# Autodesk Inventor assembly: BP-100
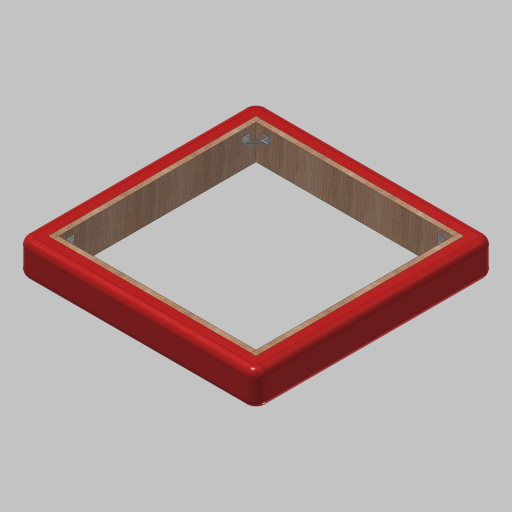
[picture p0: Inventor's stored thumbnail of the model, 512x512]
Saved by Autodesk Inventor 2023.5 (Build 275446000, 446)
## iProperties
Created: 2025-01-26
Part Number: BP-100
Document SubType Name: Assembly
Designer: slick
Author: slick
## Documents named in this file (5)
- C:\Users\slick\OneDrive\Desktop\2025-ReefScape---CAD\Bumpers\BP-100.iam
- C:\Users\slick\OneDrive\Desktop\2025-ReefScape---CAD\Bumpers\BP-001.ipt
- C:\Users\slick\OneDrive\Desktop\2025-ReefScape---CAD\Bumpers\BP-002.ipt
- C:\Users\slick\OneDrive\Desktop\2025-ReefScape---CAD\Bumpers\BP-0036.ipt
- C:\Users\slick\OneDrive\Desktop\2025-ReefScape---CAD\Bumpers\BP-004.ipt
## Components (9 placed, 4 different names)
1. BP-001:1 — Flush:1, Mate:1, Flush:5, Mate:5, Flush:7, Insert:1, Insert:2
2. BP-001:2 — Flush:2, Flush:3, Mate:2, Flush:4, Flush:6, Mate:3, Insert:5, Insert:6
3. BP-002:1 — Flush:3, Flush:6, Mate:3, Mate:4, Insert:7, Insert:8
4. BP-002:2 — Flush:1, Flush:2, Mate:1, Mate:2, Flush:4, Flush:5, Insert:3, Insert:4
5. BP-0036:1 — Mate:4, Mate:5, Flush:7
6. BP-004:1 — Insert:1, Insert:2
7. BP-004:2 — Insert:3, Insert:4
8. BP-004:3 — Insert:5, Insert:6
9. BP-004:4 — Insert:7, Insert:8
## Relationships (20: Insert 8, Flush 7, Mate 5)
- Flush:1: BP-001:1 ↔ BP-002:2
- Flush:2: BP-001:2 ↔ BP-002:2
- Flush:3: BP-001:2 ↔ BP-002:1
- Mate:1: BP-001:1 ↔ BP-002:2
- Mate:2: BP-001:2 ↔ BP-002:2
- Flush:4: BP-001:2 ↔ BP-002:2
- Flush:5: BP-001:1 ↔ BP-002:2
- Flush:6: BP-001:2 ↔ BP-002:1
- Mate:3: BP-001:2 ↔ BP-002:1
- Mate:4: BP-002:1 ↔ BP-0036:1
- Mate:5: BP-001:1 ↔ BP-0036:1
- Flush:7: BP-001:1 ↔ BP-0036:1
- Insert:1: BP-001:1 ↔ BP-004:1
- Insert:2: BP-001:1 ↔ BP-004:1
- Insert:3: BP-002:2 ↔ BP-004:2
- Insert:4: BP-002:2 ↔ BP-004:2
- Insert:5: BP-001:2 ↔ BP-004:3
- Insert:6: BP-001:2 ↔ BP-004:3
- Insert:7: BP-002:1 ↔ BP-004:4
- Insert:8: BP-002:1 ↔ BP-004:4
